# Autodesk Inventor assembly: walker with arm rest
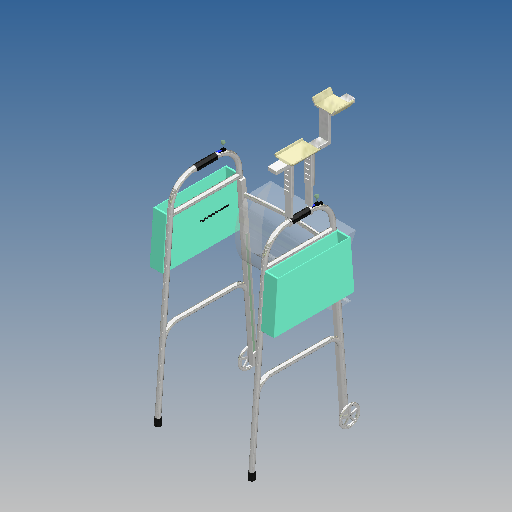
[picture p0: Inventor's stored thumbnail of the model, 512x512]
Saved by Autodesk Inventor 2021 (Build 250183000, 183)
## iProperties
Created: 2021-04-07
Part Number: walker with arm rest
Document SubType Name: Assembly
Designer: kavig
Author: kavig
## Documents named in this file (5)
- C:\Users\gurle\Downloads\assy walker.iam
- C:\Users\gurle\Downloads\walker.ipt
- C:\Users\gurle\Downloads\arm rest.ipt
- C:\Users\gurle\Downloads\arm rest base.ipt
- C:\Users\gurle\Downloads\shovel.ipt
## Components (5 placed, 4 different names)
1. walker:1 — Mate:1, Mate:2, Angle:1, Angle:2, Flush:1, Mate:7, Tangent:1, Tangent:2, Angle:3
2. arm rest base:1 — Mate:2, Angle:1, Flush:1, Mate:3, Mate:4, Mate:5
3. arm rest base:2 — Mate:1, Angle:2, Mate:6
4. arm rest:1 — Mate:3, Mate:4, Mate:5, Mate:6
5. shovel:1 — Mate:7, Tangent:1, Tangent:2, Angle:3
## Relationships (13: Mate 7, Angle 3, Tangent 2, Flush 1)
- Mate:1: walker:1 ↔ arm rest base:2
- Mate:2: walker:1 ↔ arm rest base:1
- Angle:1 (0 deg): walker:1 ↔ arm rest base:1
- Angle:2 (0 deg): walker:1 ↔ arm rest base:2
- Flush:1: walker:1 ↔ arm rest base:1
- Mate:3: arm rest base:1 ↔ arm rest:1
- Mate:4 (1.482 mm): arm rest base:1 ↔ arm rest:1
- Mate:5 (1 mm): arm rest base:1 ↔ arm rest:1
- Mate:6 (1 mm): arm rest base:2 ↔ arm rest:1
- Mate:7: walker:1 ↔ shovel:1
- Tangent:1: walker:1 ↔ shovel:1
- Tangent:2: walker:1 ↔ shovel:1
- Angle:3 (0 deg): walker:1 ↔ shovel:1
